# Autodesk Inventor assembly: Assembly1
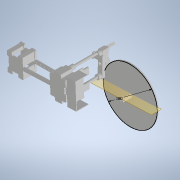
[picture p0: Inventor's stored thumbnail of the model, 180x180]
Saved by Autodesk Inventor 2022 (Build 260153000, 153)
## iProperties
Created: 2021-12-30
Part Number: Assembly1
Document SubType Name: Assembly
Designer: simon
Author: simon
## Documents named in this file (8)
- C:\Users\Uporabnik\Desktop\Simon\3d model (5)\Assembly1.iam
- C:\Users\Uporabnik\Desktop\Simon\3d model (5)\Hold of motors.ipt
- C:\Users\Uporabnik\Desktop\Simon\3d model (5)\zaponka za motor2.ipt
- C:\Users\Uporabnik\Desktop\Simon\3d model (5)\constraining plate.ipt
- C:\Users\Uporabnik\Desktop\Simon\3d model (5)\spirale.ipt
- C:\Users\Uporabnik\Desktop\Simon\3d model (5)\drzalo_vezja.ipt
- C:\Users\Uporabnik\Desktop\Simon\3d model (5)\priključek za matice.ipt
- C:\Users\Uporabnik\Desktop\Simon\3d model (5)\plošča za vrtenje.ipt
## Components (8 placed, 8 different names)
1. Hold of motors:1 — Flush:2, Flush:3, Rotational:2, Rotational:5, Mate:1, Mate:2, Flush:7
2. zaponka za motor2:1 — Flush:2, Flush:3, Mate:3, Flush:5
3. constraining plate:1 — Rotational:4, Flush:4
4. hold_rod:1 — Rotational:5
5. spirale:2 — Rotational:2, Rotational:4
6. drzalo_vezja:1 — Mate:1, Mate:2, Mate:3, Flush:6
7. priključek za matice:1 — Flush:4
8. plošča za vrtenje:1 — Flush:5, Flush:6, Flush:7
## Relationships (12: Flush 6, RevoluteJoint 3, Mate 3)
- Flush:2: Hold of motors:1 ↔ zaponka za motor2:1
- Flush:3: Hold of motors:1 ↔ zaponka za motor2:1
- Rotational:2 [RevoluteJoint]: Hold of motors:1 ↔ spirale:2
- Rotational:4 [RevoluteJoint]: constraining plate:1 ↔ spirale:2
- Rotational:5 [RevoluteJoint]: Hold of motors:1 ↔ hold_rod:1
- Mate:1: Hold of motors:1 ↔ drzalo_vezja:1
- Mate:2: Hold of motors:1 ↔ drzalo_vezja:1
- Mate:3: zaponka za motor2:1 ↔ drzalo_vezja:1
- Flush:4: constraining plate:1 ↔ priključek za matice:1
- Flush:5: zaponka za motor2:1 ↔ plošča za vrtenje:1
- Flush:6: drzalo_vezja:1 ↔ plošča za vrtenje:1
- Flush:7: Hold of motors:1 ↔ plošča za vrtenje:1
